# Autodesk Inventor assembly: AllRCUs
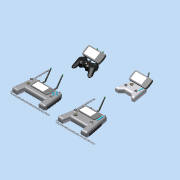
[picture p0: Inventor's stored thumbnail of the model, 180x180]
Saved by Autodesk Inventor 2011 SP1 (Build 150282100, 282)
## iProperties
Created: 2011-08-16
Part Number: AllRCUs
Document SubType Name: Assembly
Designer: dgitz
Author: dgitz
## Documents named in this file (5)
- C:\Dropbox\ICARUS\Remote Control Unit (RCU)\RCU v2\Design\AllRCUs.iam
- C:\Dropbox\ICARUS\Remote Control Unit (RCU)\RCU v2\Design\RCUv2-1Assy.iam
- C:\Dropbox\ICARUS\Remote Control Unit (RCU)\RCU v2\Design\RCUv2-2Assy.iam
- C:\Dropbox\ICARUS\Remote Control Unit (RCU)\RCU v2\Design\RCUv2-3Assy.iam
- C:\Dropbox\ICARUS\Remote Control Unit (RCU)\RCU v2\Design\RCUv2-4Assy.iam
## Components (4 placed, 4 different names)
1. RCUv2-1Assy:1 [sub-assembly] — Flush:1, Mate:1
2. RCUv2-2Assy:1 [sub-assembly] — Flush:2, Mate:2
3. RCUv2-3Assy:1 [sub-assembly] — Flush:3, Mate:3
4. RCUv2-4Assy:1 [sub-assembly] — Flush:4, Mate:4
## Relationships (8: Flush 4, Mate 4)
- Flush:1: RCUv2-1Assy:1
- Mate:1 (-101.6 mm): RCUv2-1Assy:1
- Flush:2: RCUv2-2Assy:1
- Mate:2 (254 mm): RCUv2-2Assy:1
- Flush:3: RCUv2-3Assy:1
- Mate:3 (-101.6 mm): RCUv2-3Assy:1
- Flush:4: RCUv2-4Assy:1
- Mate:4 (254 mm): RCUv2-4Assy:1
